# Autodesk Inventor assembly: Climbing Arm 1
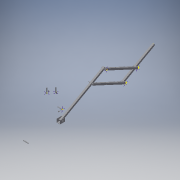
[picture p0: Inventor's stored thumbnail of the model, 180x180]
Saved by Autodesk Inventor 2016 (Build 200138000, 138)
## iProperties
Created: 2016-01-28
Part Number: Climbing Arm 1
Document SubType Name: Assembly
Designer: Jack Jaworski
Author: Jack Jaworski
## Documents named in this file (10)
- C:\Users\Admin\Desktop\Scaling Arms\Climbing Arm 1.iam
- C:\Users\Admin\Desktop\Scaling Arms\3-8 2.5 Inch Hex Bolt.ipt
- C:\Users\Admin\Desktop\Scaling Arms\3-8 Inch Hex Nut.ipt
- C:\Users\Admin\Desktop\Scaling Arms\1x1 16th Inch Aluminum Tube - Custom for Lift Arms.ipt
- C:\Users\Admin\Desktop\Scaling Arms\1x1 8th Inch Aluminum Tube Custom Lift Arms.ipt
- C:\Users\Admin\Desktop\Scaling Arms\Scaling Arms Mounting Bracket.ipt
- C:\Users\Admin\Desktop\Scaling Arms\3 Inch Hex Chafter.ipt
- C:\Users\Admin\Desktop\Scaling Arms\3 8th Inch Flanged Bearing.ipt
- C:\Users\Admin\Downloads\217-2733-STEP\3-8th inch hex bearing small.ipt
- C:\Users\Admin\Desktop\Scaling Arms\3 inch round Shaft 2.ipt
## Components (24 placed, 9 different names)
1. 3-8 2.5 Inch Hex Bolt:1
2. 3-8 2.5 Inch Hex Bolt:2 — Rotational:6
3. 3-8 2.5 Inch Hex Bolt:4 — Rotational:5
4. 3-8 2.5 Inch Hex Bolt:6 — Rotational:13
5. 3-8 Inch Hex Nut:1
6. 3-8 Inch Hex Nut:2 — Rotational:9
7. 3-8 Inch Hex Nut:6 — Rotational:10
8. 3-8 Inch Hex Nut:7 — Rotational:15
9. 1x1 16th Inch Aluminum Tube - Custom for Lift Arms:1 — Rotational:6, Rotational:7, Rotational:21
10. 1x1 16th Inch Aluminum Tube - Custom for Lift Arms:2 — Rotational:5, Rotational:8, Rotational:11, Rotational:13
11. 1x1 16th Inch Aluminum Tube - Custom for Lift Arms:3 — Rotational:7, Rotational:8, Rotational:9, Rotational:10
12. 1x1 8th Inch Aluminum Tube Custom Lift Arms:1 — Rotational:11, Rotational:15, Slider:1, Flush:1, Mate:1, Rotational:19, Rotational:20
13. 3 Inch Hex Chafter:1 — Slider:1, Slider:2, Flush:1
14. 3 8th Inch Flanged Bearing:1 — Rotational:18, Mate:1
15. 3 8th Inch Flanged Bearing:2 — Rotational:17, Slider:2
16. 3-8 2.5 Inch Hex Bolt:7
17. 3-8 2.5 Inch Hex Bolt:8
18. 3-8 Inch Hex Nut:8
19. 3-8 Inch Hex Nut:9
20. Scaling Arms Mounting Bracket:1 — Rotational:17, Rotational:18
21. 3 Inch Hex Chafter:2
22. 3-8th inch hex bearing small:1 — Rotational:19
23. 3-8th inch hex bearing small:2 — Rotational:20, Cylindrical:1
24. 3 inch round Shaft 2:1 — Cylindrical:1, Rotational:21
## Relationships (19: RevoluteJoint 14, TranslationJoint 2, Flush 1, Mate 1, CylindricalJoint 1)
- Rotational:5 [RevoluteJoint]: 3-8 2.5 Inch Hex Bolt:4 ↔ 1x1 16th Inch Aluminum Tube - Custom for Lift Arms:2
- Rotational:6 [RevoluteJoint]: 3-8 2.5 Inch Hex Bolt:2 ↔ 1x1 16th Inch Aluminum Tube - Custom for Lift Arms:1
- Rotational:7 [RevoluteJoint]: 1x1 16th Inch Aluminum Tube - Custom for Lift Arms:1 ↔ 1x1 16th Inch Aluminum Tube - Custom for Lift Arms:3
- Rotational:8 [RevoluteJoint]: 1x1 16th Inch Aluminum Tube - Custom for Lift Arms:2 ↔ 1x1 16th Inch Aluminum Tube - Custom for Lift Arms:3
- Rotational:9 [RevoluteJoint]: 3-8 Inch Hex Nut:2 ↔ 1x1 16th Inch Aluminum Tube - Custom for Lift Arms:3
- Rotational:10 [RevoluteJoint]: 3-8 Inch Hex Nut:6 ↔ 1x1 16th Inch Aluminum Tube - Custom for Lift Arms:3
- Rotational:11 [RevoluteJoint]: 1x1 16th Inch Aluminum Tube - Custom for Lift Arms:2 ↔ 1x1 8th Inch Aluminum Tube Custom Lift Arms:1
- Rotational:13 [RevoluteJoint]: 3-8 2.5 Inch Hex Bolt:6 ↔ 1x1 16th Inch Aluminum Tube - Custom for Lift Arms:2
- Rotational:15 [RevoluteJoint]: 3-8 Inch Hex Nut:7 ↔ 1x1 8th Inch Aluminum Tube Custom Lift Arms:1
- Slider:1 [TranslationJoint]: 1x1 8th Inch Aluminum Tube Custom Lift Arms:1 ↔ 3 Inch Hex Chafter:1
- Rotational:17 [RevoluteJoint]: 3 8th Inch Flanged Bearing:2 ↔ Scaling Arms Mounting Bracket:1
- Rotational:18 [RevoluteJoint]: 3 8th Inch Flanged Bearing:1 ↔ Scaling Arms Mounting Bracket:1
- Slider:2 [TranslationJoint]: 3 Inch Hex Chafter:1 ↔ 3 8th Inch Flanged Bearing:2
- Flush:1 (-25.4 mm): 1x1 8th Inch Aluminum Tube Custom Lift Arms:1 ↔ 3 Inch Hex Chafter:1
- Mate:1 (6.35 mm): 1x1 8th Inch Aluminum Tube Custom Lift Arms:1 ↔ 3 8th Inch Flanged Bearing:1
- Rotational:19 [RevoluteJoint]: 1x1 8th Inch Aluminum Tube Custom Lift Arms:1 ↔ 3-8th inch hex bearing small:1
- Rotational:20 [RevoluteJoint]: 1x1 8th Inch Aluminum Tube Custom Lift Arms:1 ↔ 3-8th inch hex bearing small:2
- Cylindrical:1: 3-8th inch hex bearing small:2 ↔ 3 inch round Shaft 2:1
- Rotational:21 [RevoluteJoint]: 1x1 16th Inch Aluminum Tube - Custom for Lift Arms:1 ↔ 3 inch round Shaft 2:1
